# Autodesk Inventor assembly: 1400_DC Coil_V1
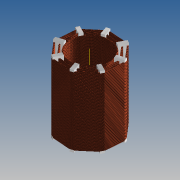
[picture p0: Inventor's stored thumbnail of the model, 180x180]
Saved by Autodesk Inventor 2020 (Build 240168000, 168)
## iProperties
Created: 2019-11-14
Part Number: 1400_DC Coil_V1
Document SubType Name: Assembly
Designer: RFLab
Author: RFLab
## Documents named in this file (6)
- C:\Users\RFLab\Dropbox\MPI Group Folder\MPS\Inventor_Parts\Parts Numbered - OSMPI\1xxx_Transmit Assembly\14xx_Bias Coils\1400_DC Coil_V1.iam
- C:\Users\RFLab\Dropbox\MPI Group Folder\MPS\Inventor_Parts\Coils\DC_Bias\2019_11_14_1stlayer.ipt
- C:\Users\RFLab\Dropbox\MPI Group Folder\MPS\Inventor_Parts\Coils\DC_Bias\2019_11_11_spacer_dcbiasingcoil_1st.ipt
- C:\Users\RFLab\Dropbox\MPI Group Folder\MPS\Inventor_Parts\Coils\DC_Bias\2019_11_14_2ndlayer.ipt
- C:\Users\RFLab\Dropbox\MPI Group Folder\MPS\Inventor_Parts\Coils\DC_Bias\2019_11_11_spacer_dcbiasingcoil_2nd.ipt
- C:\Users\RFLab\Dropbox\MPI Group Folder\MPS\Inventor_Parts\Coils\DC_Bias\2019_11_14_3rdlayer.ipt
## Components (5 placed, 5 different names)
1. 2019_11_14_1stlayer:1 — Mate:1, Angle:1, Mate:3, Mate:4, Mate:6, Mate:8
2. 2019_11_11_spacer_dcbiasingcoil_1st:1 — Mate:4, Mate:5, Mate:7, Flush:1, Flush:2, Angle:3
3. 2019_11_14_2ndlayer:1 — Mate:6, Mate:7, Angle:2, Angle:3, Angle:4
4. 2019_11_11_spacer_dcbiasingcoil_2nd:1 — Mate:8, Flush:1, Angle:2, Flush:2, Mate:9, Mate:10
5. 2019_11_14_3rdlayer:1 — Mate:9, Mate:10, Angle:4
## Relationships (15: Mate 9, Angle 4, Flush 2)
- Mate:1: 2019_11_14_1stlayer:1
- Angle:1 (0 deg): 2019_11_14_1stlayer:1
- Mate:3: 2019_11_14_1stlayer:1
- Mate:4: 2019_11_14_1stlayer:1 ↔ 2019_11_11_spacer_dcbiasingcoil_1st:1
- Mate:5 (-3.45 mm): 2019_11_11_spacer_dcbiasingcoil_1st:1
- Mate:6: 2019_11_14_1stlayer:1 ↔ 2019_11_14_2ndlayer:1
- Mate:7 (0.45 mm): 2019_11_11_spacer_dcbiasingcoil_1st:1 ↔ 2019_11_14_2ndlayer:1
- Mate:8: 2019_11_14_1stlayer:1 ↔ 2019_11_11_spacer_dcbiasingcoil_2nd:1
- Flush:1: 2019_11_11_spacer_dcbiasingcoil_1st:1 ↔ 2019_11_11_spacer_dcbiasingcoil_2nd:1
- Angle:2 (0 deg): 2019_11_14_2ndlayer:1 ↔ 2019_11_11_spacer_dcbiasingcoil_2nd:1
- Flush:2: 2019_11_11_spacer_dcbiasingcoil_1st:1 ↔ 2019_11_11_spacer_dcbiasingcoil_2nd:1
- Mate:9: 2019_11_11_spacer_dcbiasingcoil_2nd:1 ↔ 2019_11_14_3rdlayer:1
- Mate:10 (0.45 mm): 2019_11_11_spacer_dcbiasingcoil_2nd:1 ↔ 2019_11_14_3rdlayer:1
- Angle:3 (0 deg): 2019_11_11_spacer_dcbiasingcoil_1st:1 ↔ 2019_11_14_2ndlayer:1
- Angle:4 (0 deg): 2019_11_14_2ndlayer:1 ↔ 2019_11_14_3rdlayer:1
